# Autodesk Inventor assembly: sandbox
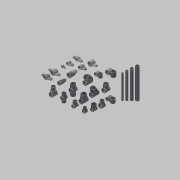
[picture p0: Inventor's stored thumbnail of the model, 180x180]
Saved by Autodesk Inventor 2019.4 (Build 234330000, 330)
## iProperties
RuleStatus: InUse
Created: 2020-04-27
Part Number: sandbox
Document SubType Name: Assembly
Designer: Hannah
Author: Hannah
## Documents named in this file (28)
- \\Mac\Home\Documents\GitHub\AdjustaBike-2.0\CAD\sandbox.iam
- \\Mac\Home\Documents\GitHub\AdjustaBike-2.0\CAD\10-65.ipt
- \\Mac\Home\Documents\GitHub\AdjustaBike-2.0\CAD\10-67.ipt
- \\Mac\Home\Documents\GitHub\AdjustaBike-2.0\CAD\10-76.ipt
- \\Mac\Home\Documents\GitHub\AdjustaBike-2.0\CAD\45-76.ipt
- \\Mac\Home\Documents\GitHub\AdjustaBike-2.0\CAD\86-7.ipt
- \\Mac\Home\Documents\GitHub\AdjustaBike-2.0\CAD\329-7.ipt
- \\Mac\Home\Documents\GitHub\AdjustaBike-2.0\CAD\L10-6.ipt
- \\Mac\Home\Documents\GitHub\AdjustaBike-2.0\CAD\L10-7.ipt
- \\Mac\Home\Documents\GitHub\AdjustaBike-2.0\CAD\L26-6.ipt
- \\Mac\Home\Documents\GitHub\AdjustaBike-2.0\CAD\L26-7.ipt
- \\Mac\Home\Documents\GitHub\AdjustaBike-2.0\CAD\L29-7.ipt
- \\Mac\Home\Documents\GitHub\AdjustaBike-2.0\CAD\L45-6.ipt
- \\Mac\Home\Documents\GitHub\AdjustaBike-2.0\CAD\L45-7.ipt
- \\Mac\Home\Documents\GitHub\AdjustaBike-2.0\CAD\L114-7.ipt
- \\Mac\Home\Documents\GitHub\AdjustaBike-2.0\CAD\LF50-6.ipt
- \\Mac\Home\Documents\GitHub\AdjustaBike-2.0\CAD\LF50-7.ipt
- \\Mac\Home\Documents\GitHub\AdjustaBike-2.0\CAD\LM50-6.ipt
- \\Mac\Home\Documents\GitHub\AdjustaBike-2.0\CAD\LM50-7.ipt
- \\Mac\Home\Documents\GitHub\AdjustaBike-2.0\CAD\LM51-6.ipt
- \\Mac\Home\Documents\GitHub\AdjustaBike-2.0\CAD\LM51-7.ipt
- \\Mac\Home\Documents\GitHub\AdjustaBike-2.0\CAD\M50-4.ipt
- \\Mac\Home\Documents\GitHub\AdjustaBike-2.0\CAD\M50-5.ipt
- \\Mac\Home\Documents\GitHub\AdjustaBike-2.0\CAD\M51-5.ipt
- \\Mac\Home\Documents\GitHub\AdjustaBike-2.0\CAD\tube-02.ipt
- \\Mac\Home\Documents\GitHub\AdjustaBike-2.0\CAD\tube-03.ipt
- \\Mac\Home\Documents\GitHub\AdjustaBike-2.0\CAD\tube-05.ipt
- \\Mac\Home\Documents\GitHub\AdjustaBike-2.0\CAD\tube-06.ipt
## Components (27 placed, 27 different names)
1. 10-65:1
2. 10-67:1
3. 10-76:1
4. 45-76:1
5. 86-7:1
6. 329-7:1
7. L10-6:1
8. L10-7:1
9. L26-6:1
10. L26-7:1
11. L29-7:1
12. L45-6:1
13. L45-7:1
14. L114-7:1
15. LF50-6:1
16. LF50-7:1
17. LM50-6:1
18. LM50-7:1
19. LM51-6:1
20. LM51-7:1
21. M50-4:1
22. M50-5:1
23. M51-5:1
24. tube-02:1
25. tube-03:1
26. tube-05:1
27. tube-06:1
## Named parameters: La = 300 mm, Lb = 325 mm, Lc = 350 mm, Ld = 375 mm, Sa = 4, Sb = 5, Sc = 6, Sd = 7
